# Autodesk Inventor assembly: RubberFootAssembly
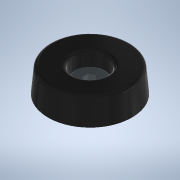
[picture p0: Inventor's stored thumbnail of the model, 180x180]
Saved by Autodesk Inventor 2022 (Build 260153000, 153)
## iProperties
Created: 2021-11-08
Part Number: RubberFootAssembly
Document SubType Name: Assembly
Designer: FabLab
Author: FabLab
## Documents named in this file (4)
- C:\Users\JK\Documents\Inventor\UTM\RubberFootAssembly.iam
- C:\Users\JK\Documents\Inventor\UTM\RubberFoot.ipt
- C:\Users\JK\Documents\Inventor\UTM\TuercaTM5Perfil2020.ipt
- C:\Users\JK\Documents\Inventor\UTM\PernoM5x8Plano.ipt
## Components (3 placed, 3 different names)
1. RubberFoot:1 — Coincidencia:1, Coincidencia:2, Coincidencia:3, Coincidencia:4, Ángulo:1
2. TuercaTM5Perfil2020:1 — Coincidencia:1, Coincidencia:4, Ángulo:1
3. PernoM5x8Plano:1 — Coincidencia:2, Coincidencia:3
## Relationships (5: Mate 4, Angle 1)
- Coincidencia:1 [Mate]: RubberFoot:1 ↔ TuercaTM5Perfil2020:1
- Coincidencia:2 [Mate]: RubberFoot:1 ↔ PernoM5x8Plano:1
- Coincidencia:3 [Mate]: RubberFoot:1 ↔ PernoM5x8Plano:1
- Coincidencia:4 [Mate] (1 mm): RubberFoot:1 ↔ TuercaTM5Perfil2020:1
- Ángulo:1 [Angle] (0 deg): RubberFoot:1 ↔ TuercaTM5Perfil2020:1
